# Autodesk Inventor assembly: Mecanismo Prueba
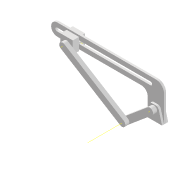
[picture p0: Inventor's stored thumbnail of the model, 180x180]
Saved by Autodesk Inventor 2021 (Build 250183000, 183)
## iProperties
Created: 2021-07-04
Part Number: Mecanismo Prueba
Document SubType Name: Assembly
Designer: Santiago
Author: Santiago
## Documents named in this file (5)
- C:\Users\user\Desktop\Ingeniería Mecánica UN\6. Sexto Semestre\Métodos Numéricos\ProyectoMetodos\Simulación Inventor\Mecanismo Prueba.iam
- C:\Users\user\Desktop\Ingeniería Mecánica UN\6. Sexto Semestre\Métodos Numéricos\ProyectoMetodos\Simulación Inventor\Acoplador.ipt
- C:\Users\user\Desktop\Ingeniería Mecánica UN\6. Sexto Semestre\Métodos Numéricos\ProyectoMetodos\Simulación Inventor\Bancada.ipt
- C:\Users\user\Desktop\Ingeniería Mecánica UN\6. Sexto Semestre\Métodos Numéricos\ProyectoMetodos\Simulación Inventor\Corredera.ipt
- C:\Users\user\Desktop\Ingeniería Mecánica UN\6. Sexto Semestre\Métodos Numéricos\ProyectoMetodos\Simulación Inventor\Manivela.ipt
## Components (4 placed, 4 different names)
1. Acoplador:1 — Mate:3, Mate:5, Mate:8, Mate:9
2. Bancada:1 — Mate:1, Mate:2, Mate:7
3. Corredera:1 — Mate:5, Mate:7, Mate:9
4. Manivela:1 — Mate:1, Mate:2, Mate:3, Mate:8
## Relationships (7: Mate 7)
- Mate:1: Bancada:1 ↔ Manivela:1
- Mate:2: Bancada:1 ↔ Manivela:1
- Mate:3: Acoplador:1 ↔ Manivela:1
- Mate:5: Acoplador:1 ↔ Corredera:1
- Mate:7: Bancada:1 ↔ Corredera:1
- Mate:8: Acoplador:1 ↔ Manivela:1
- Mate:9: Acoplador:1 ↔ Corredera:1
